# Autodesk Inventor assembly: 784002_Header Right Angle 21x3 .1in
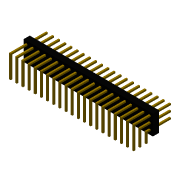
[picture p0: Inventor's stored thumbnail of the model, 180x180]
Saved by Autodesk Inventor 2015 (Build 190159000, 159)
## iProperties
Created: 2014-08-20
Part Number: 784002_Header Right Angle 21x3 .1in
Document SubType Name: Assembly
Designer: david
Author: david
## Documents named in this file (2)
- C:\SharedDrive\Dropbox\FAST Robotics\Products\818004_Power Shield\MECH\810004_Power Shield\784002_Header Right Angle 21x3 .1in.iam
- C:\SharedDrive\Dropbox\FAST Robotics\Products\818004_Power Shield\MECH\810004_Power Shield\HeaderRight3.ipt
## Components (21 placed, 1 different names)
1. HeaderRight3:22 — Mate:1
2. HeaderRight3:23
3. HeaderRight3:24
4. HeaderRight3:25
5. HeaderRight3:26
6. HeaderRight3:27
7. HeaderRight3:28
8. HeaderRight3:29
9. HeaderRight3:30
10. HeaderRight3:31
11. HeaderRight3:32
12. HeaderRight3:33
13. HeaderRight3:34
14. HeaderRight3:35
15. HeaderRight3:36
16. HeaderRight3:37
17. HeaderRight3:38
18. HeaderRight3:39
19. HeaderRight3:40
20. HeaderRight3:41
21. HeaderRight3:42
## Component patterns: (21 elements, first: HeaderRight3:22)
## Relationships (1: Mate 1)
- Mate:1: HeaderRight3:22
